# Autodesk Inventor assembly: Assembly2finally
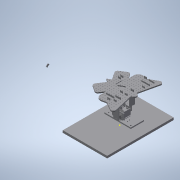
[picture p0: Inventor's stored thumbnail of the model, 180x180]
Saved by Autodesk Inventor 2020 (Build 240168000, 168)
## iProperties
Created: 2020-02-29
Part Number: Assembly2finally
Document SubType Name: Assembly
Designer: Hp
Author: Hp
## Documents named in this file (15)
- C:\Users\Hp\Desktop\siri revant\final3ddiagrams\Assembly2finally.iam
- C:\Users\Hp\Desktop\siri revant\final3ddiagrams\baseforclamp.ipt
- C:\Users\Hp\Desktop\siri revant\final3ddiagrams\basestand.ipt
- C:\Users\Hp\Desktop\siri revant\final3ddiagrams\clampforplatform.ipt
- C:\Users\Hp\Desktop\siri revant\final3ddiagrams\Lclamp1.ipt
- C:\Users\Hp\Desktop\siri revant\final3ddiagrams\Lclamp2.ipt
- C:\Users\Hp\Desktop\siri revant\final3ddiagrams\openslotforclamp.ipt
- C:\Users\Hp\Desktop\siri revant\final3ddiagrams\Part5.ipt
- C:\Users\Hp\Desktop\siri revant\final3ddiagrams\servostand.ipt
- C:\Users\Hp\Desktop\siri revant\final3ddiagrams\sidestandforservoclamp.ipt
- C:\Users\Hp\Desktop\siri revant\final3ddiagrams\HS-225MG.ipt
- C:\Users\Hp\Desktop\siri revant\final3ddiagrams\Ruderhorn.ipt
- C:\Users\Hp\Desktop\siri revant\final3ddiagrams\Part6.ipt
- C:\Users\Hp\Desktop\siri revant\final3ddiagrams\Bocks.ipt
- C:\Users\Hp\Desktop\siri revant\final3ddiagrams\Butterfly(my own.3).ipt
## Components (46 placed, 14 different names)
1. baseforclamp:1 — Rotational:2, Rigid:1, Rotational:7
2. basestand:1 — Rotational:1
3. clampforplatform:1 — Rotational:7, Rotational:8
4. Lclamp1:1 — Rotational:6, Rotational:9
5. openslotforclamp:1 — Rigid:1, Rotational:3, Rotational:4
6. Part5:1
7. servostand:1 — Rotational:1, Rotational:2, Rigid:2
8. sidestandforservoclamp:1 — Rotational:4
9. sidestandforservoclamp:2 — Rotational:3
10. HS-225MG:1 — Rigid:2, Rotational:5
11. Ruderhorn:1 — Rotational:5, Rotational:6
12. Lclamp1:2 — Rotational:8
13. Part6:1
14. Lclamp2:1 — Rotational:9, Rotational:10
15. baseforclamp:2 — Rotational:10, Rotational:11, Rotational:14, Rotational:16
16. clampforplatform:2 — Rotational:16, Rotational:18
17. Lclamp1:3 — Rotational:18, Rigid:3
18. Lclamp2:3 — Rigid:3
19. openslotforclamp:2 — Rotational:11, Rotational:12, Rotational:13
20. Part5:2
21. sidestandforservoclamp:3 — Rotational:12
22. sidestandforservoclamp:4 — Rotational:13
23. HS-225MG:2 — Rotational:14, Rotational:15
24. Ruderhorn:2 — Rotational:15, Rotational:17
25. Lclamp1:4 — Rotational:17
26. Bocks:1 — Rotational:19
27. Butterfly(my own.3):1 — Rotational:19
28. Bocks:2
29. Bocks:3
30. Bocks:4
31. Bocks:5
32. Bocks:6
33. Bocks:7
34. Bocks:8
35. Bocks:9
36. Bocks:10
37. Bocks:11
38. Bocks:12
39. Bocks:13
40. Bocks:14
41. Bocks:15
42. Bocks:16
43. Bocks:17
44. Bocks:18
45. Bocks:19
46. Bocks:20
## Relationships (22: RevoluteJoint 19, WeldJoint 3)
- Rotational:1 [RevoluteJoint] (5 mm): basestand:1 ↔ servostand:1
- Rotational:2 [RevoluteJoint] (5 mm): baseforclamp:1 ↔ servostand:1
- Rigid:1 [WeldJoint]: baseforclamp:1 ↔ openslotforclamp:1
- Rotational:3 [RevoluteJoint]: openslotforclamp:1 ↔ sidestandforservoclamp:2
- Rotational:4 [RevoluteJoint]: openslotforclamp:1 ↔ sidestandforservoclamp:1
- Rigid:2 [WeldJoint] (5 mm): servostand:1 ↔ HS-225MG:1
- Rotational:5 [RevoluteJoint]: HS-225MG:1 ↔ Ruderhorn:1
- Rotational:6 [RevoluteJoint] (-2 mm): Lclamp1:1 ↔ Ruderhorn:1
- Rotational:7 [RevoluteJoint] (5 mm): baseforclamp:1 ↔ clampforplatform:1
- Rotational:8 [RevoluteJoint] (2 mm): clampforplatform:1 ↔ Lclamp1:2
- Rotational:9 [RevoluteJoint]: Lclamp1:1 ↔ Lclamp2:1
- Rotational:10 [RevoluteJoint] (2 mm): Lclamp2:1 ↔ baseforclamp:2
- Rotational:11 [RevoluteJoint]: baseforclamp:2 ↔ openslotforclamp:2
- Rotational:12 [RevoluteJoint]: openslotforclamp:2 ↔ sidestandforservoclamp:3
- Rotational:13 [RevoluteJoint]: openslotforclamp:2 ↔ sidestandforservoclamp:4
- Rotational:14 [RevoluteJoint]: baseforclamp:2 ↔ HS-225MG:2
- Rotational:15 [RevoluteJoint]: HS-225MG:2 ↔ Ruderhorn:2
- Rotational:16 [RevoluteJoint] (2 mm): baseforclamp:2 ↔ clampforplatform:2
- Rotational:17 [RevoluteJoint] (-3 mm): Ruderhorn:2 ↔ Lclamp1:4
- Rotational:18 [RevoluteJoint] (-2 mm): clampforplatform:2 ↔ Lclamp1:3
- Rigid:3 [WeldJoint]: Lclamp1:3 ↔ Lclamp2:3
- Rotational:19 [RevoluteJoint]: Bocks:1 ↔ Butterfly(my own.3):1
